# Autodesk Inventor assembly: Spring apparatus assembly V2
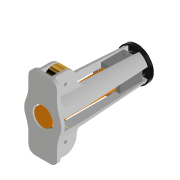
[picture p0: Inventor's stored thumbnail of the model, 180x180]
Saved by Autodesk Inventor 2021.3 (Build 253353000, 353)
## iProperties
Created: 2022-07-02
Part Number: Spring apparatus assembly V2
Document SubType Name: Assembly
Designer: david
Author: david
## Documents named in this file (6)
- C:\Users\david\Desktop\ChalkBot\Spring apparatus assembly V2.iam
- C:\Users\david\Desktop\ChalkBot\CF Spring with hole.ipt
- C:\Users\david\Desktop\ChalkBot\Cap V2 (App V5).ipt
- C:\Users\david\Desktop\ChalkBot\Slider V4-2 (spring with hole).ipt
- C:\Users\david\Desktop\ChalkBot\Spring apparatus V5.ipt
- C:\Users\david\Desktop\ChalkBot\Chalk.ipt
## Components (6 placed, 5 different names)
1. CF Spring with hole:1 — Cylindrical:3
2. CF Spring with hole:2 — Cylindrical:1
3. Cap V2 (App V5):1 — Rigid:1
4. Slider V4-2 (spring with hole):1 — Cylindrical:2, Mate:1
5. Spring apparatus V5:1 — Cylindrical:1, Cylindrical:2, Cylindrical:3, Rigid:1
6. Chalk:1 — Mate:1
## Relationships (5: CylindricalJoint 3, WeldJoint 1, Mate 1)
- Cylindrical:1: CF Spring with hole:2 ↔ Spring apparatus V5:1
- Cylindrical:2: Slider V4-2 (spring with hole):1 ↔ Spring apparatus V5:1
- Cylindrical:3: CF Spring with hole:1 ↔ Spring apparatus V5:1
- Rigid:1 [WeldJoint]: Cap V2 (App V5):1 ↔ Spring apparatus V5:1
- Mate:1: Slider V4-2 (spring with hole):1 ↔ Chalk:1
